# Autodesk Inventor assembly: Коробка с крышкой
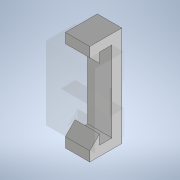
[picture p0: Inventor's stored thumbnail of the model, 180x180]
Saved by Autodesk Inventor 2020 (Build 240168000, 168)
## iProperties
Created: 2021-04-26
Part Number: Коробка с крышкой
Document SubType Name: Assembly
Designer: Антон
Author: Антон
## Documents named in this file (3)
- D:\Project\Robots\RRO 2021\Test\Коробка с крышкой.iam
- D:\Project\Robots\RRO 2021\Test\Тестовая коробка.ipt
- D:\Project\Robots\RRO 2021\Test\Тестовая крышка.ipt
## Components (2 placed, 2 different names)
1. Тестовая коробка:1 — Жесткий:1
2. Тестовая крышка:1 — Жесткий:1
## Relationships (1: WeldJoint 1)
- Жесткий:1 [WeldJoint]: Тестовая коробка:1 ↔ Тестовая крышка:1
